# Autodesk Inventor assembly: main_assembly
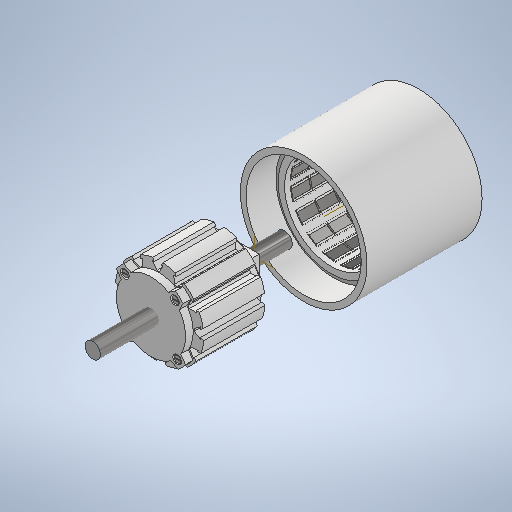
[picture p0: Inventor's stored thumbnail of the model, 512x512]
Saved by Autodesk Inventor 2025 (Build 290162000, 162)
## iProperties
Created: 2026-08-03
Part Number: main_assembly
Document SubType Name: Assembly
Designer: zzapa
Author: zzapa
## Documents named in this file (11)
- C:\Users\zzapa\Desktop\Projekty\elektronika\engine-project\model\assemblies\main_assembly.iam
- C:\Users\zzapa\Desktop\Projekty\elektronika\engine-project\model\parts\stator_metal.ipt
- C:\Users\zzapa\Desktop\Projekty\elektronika\engine-project\model\assemblies\magnet_ring_assembly.iam
- C:\Users\zzapa\Desktop\Projekty\elektronika\engine-project\model\parts\casing_cylindrical.ipt
- C:\Users\zzapa\Desktop\Projekty\elektronika\engine-project\model\parts\rotor_plastic.ipt
- C:\Users\zzapa\Desktop\Projekty\elektronika\engine-project\model\assemblies\rotor_core.iam
- C:\Users\zzapa\Desktop\Projekty\elektronika\engine-project\model\parts\shaft.ipt
- C:\Users\zzapa\Documents\Inventor\Content Center Files\R2025\pl-PL\GB 809-88 A\Nut GB 809 A M2,5 x 6.ipt
- C:\Users\zzapa\Desktop\Projekty\elektronika\engine-project\model\parts\shaft_lock_1.ipt
- C:\Users\zzapa\Desktop\Projekty\elektronika\engine-project\model\parts\shaft_lock_2.ipt
- C:\Users\zzapa\Documents\Inventor\Content Center Files\R2025\pl-PL\CNS 4355\CNS 4355 - M 2 x 6.ipt
## Components (16 placed, 10 different names)
1. stator_metal:1 — Zestawiające:1, Kątowe:1
2. magnet_ring_assembly:1 [sub-assembly] — Zestawiające:2
3. casing_cylindrical:1 — Zestawiające:3, Kątowe:2
4. rotor_plastic:1 — Zestawiające:4, Zestawiające:7, Zestawiające:8, Zestawiające:9, Zestawiające:10, Równoległe:1, Równoległe:2, Równoległe:3, Równoległe:4, Zestawiające:12, Kątowe:8, Zestawiające:16, Zestawiające:18
5. rotor_core:1 [sub-assembly] — Zestawiające:5, Zestawiające:17, Zestawiające:19
6. shaft:1 — Zestawiające:6, Zestawiające:15
7. Nut GB/T 809-1988 Type A M2,5x6:1 — Kątowe:3, Zestawiające:7, Równoległe:3
8. Nut GB/T 809-1988 Type A M2,5x6:2 — Kątowe:4, Zestawiające:9, Równoległe:1
9. Nut GB/T 809-1988 Type A M2,5x6:3 — Kątowe:5, Zestawiające:8, Równoległe:2
10. Nut GB/T 809-1988 Type A M2,5x6:4 — Kątowe:6, Zestawiające:10, Równoległe:4
11. shaft_lock_1:1 — Zestawiające:12, Kątowe:7, Zestawiające:17, Zestawiające:18
12. shaft_lock_2:1 — Zestawiające:15, Zestawiające:16, Zestawiające:19, Zestawiające:20, Zestawiające:21, Zestawiające:22, Zestawiające:23, Zestawiające:24, Zestawiające:25, Zestawiające:26, Zestawiające:27
13. CNS 4355 M 2 x 6:1 — Zestawiające:23, Kątowe:9, Zestawiające:27
14. CNS 4355 M 2 x 6:2 — Zestawiające:21, Kątowe:10, Zestawiające:25
15. CNS 4355 M 2 x 6:3 — Zestawiające:22, Kątowe:11, Zestawiające:26
16. CNS 4355 M 2 x 6:4 — Zestawiające:20, Kątowe:12, Zestawiające:24
## Relationships (40: Mate 24, Angle 12, Flush 4)
- Zestawiające:1 [Mate]: stator_metal:1
- Kątowe:1 [Angle] (0 deg): stator_metal:1
- Zestawiające:2 [Mate]: magnet_ring_assembly:1
- Zestawiające:3 [Mate]: casing_cylindrical:1
- Kątowe:2 [Angle] (0 deg): casing_cylindrical:1
- Zestawiające:4 [Mate]: rotor_plastic:1
- Zestawiające:5 [Mate]: rotor_core:1
- Zestawiające:6 [Mate]: shaft:1
- Kątowe:3 [Angle] (0 deg): Nut GB/T 809-1988 Type A M2,5x6:1
- Kątowe:4 [Angle] (0 deg): Nut GB/T 809-1988 Type A M2,5x6:2
- Kątowe:5 [Angle] (0 deg): Nut GB/T 809-1988 Type A M2,5x6:3
- Kątowe:6 [Angle] (0 deg): Nut GB/T 809-1988 Type A M2,5x6:4
- Zestawiające:7 [Mate]: rotor_plastic:1 ↔ Nut GB/T 809-1988 Type A M2,5x6:1
- Zestawiające:8 [Mate]: rotor_plastic:1 ↔ Nut GB/T 809-1988 Type A M2,5x6:3
- Zestawiające:9 [Mate]: rotor_plastic:1 ↔ Nut GB/T 809-1988 Type A M2,5x6:2
- Zestawiające:10 [Mate]: rotor_plastic:1 ↔ Nut GB/T 809-1988 Type A M2,5x6:4
- Równoległe:1 [Flush]: rotor_plastic:1 ↔ Nut GB/T 809-1988 Type A M2,5x6:2
- Równoległe:2 [Flush]: rotor_plastic:1 ↔ Nut GB/T 809-1988 Type A M2,5x6:3
- Równoległe:3 [Flush]: rotor_plastic:1 ↔ Nut GB/T 809-1988 Type A M2,5x6:1
- Równoległe:4 [Flush]: rotor_plastic:1 ↔ Nut GB/T 809-1988 Type A M2,5x6:4
- Zestawiające:12 [Mate]: rotor_plastic:1 ↔ shaft_lock_1:1
- Kątowe:7 [Angle] (0 deg): shaft_lock_1:1
- Kątowe:8 [Angle] (27.5 deg): rotor_plastic:1
- Zestawiające:15 [Mate]: shaft:1 ↔ shaft_lock_2:1
- Zestawiające:16 [Mate]: rotor_plastic:1 ↔ shaft_lock_2:1
- Zestawiające:17 [Mate]: rotor_core:1 ↔ shaft_lock_1:1
- Zestawiające:18 [Mate]: rotor_plastic:1 ↔ shaft_lock_1:1
- Zestawiające:19 [Mate]: rotor_core:1 ↔ shaft_lock_2:1
- Zestawiające:20 [Mate]: shaft_lock_2:1 ↔ CNS 4355 M 2 x 6:4
- Zestawiające:21 [Mate]: shaft_lock_2:1 ↔ CNS 4355 M 2 x 6:2
- Zestawiające:22 [Mate]: shaft_lock_2:1 ↔ CNS 4355 M 2 x 6:3
- Zestawiające:23 [Mate]: shaft_lock_2:1 ↔ CNS 4355 M 2 x 6:1
- Kątowe:9 [Angle] (0 deg): CNS 4355 M 2 x 6:1
- Kątowe:10 [Angle] (0 deg): CNS 4355 M 2 x 6:2
- Kątowe:11 [Angle] (0 deg): CNS 4355 M 2 x 6:3
- Kątowe:12 [Angle] (0 deg): CNS 4355 M 2 x 6:4
- Zestawiające:24 [Mate]: shaft_lock_2:1 ↔ CNS 4355 M 2 x 6:4
- Zestawiające:25 [Mate]: shaft_lock_2:1 ↔ CNS 4355 M 2 x 6:2
- Zestawiające:26 [Mate]: shaft_lock_2:1 ↔ CNS 4355 M 2 x 6:3
- Zestawiające:27 [Mate]: shaft_lock_2:1 ↔ CNS 4355 M 2 x 6:1
